# Autodesk Inventor assembly: case
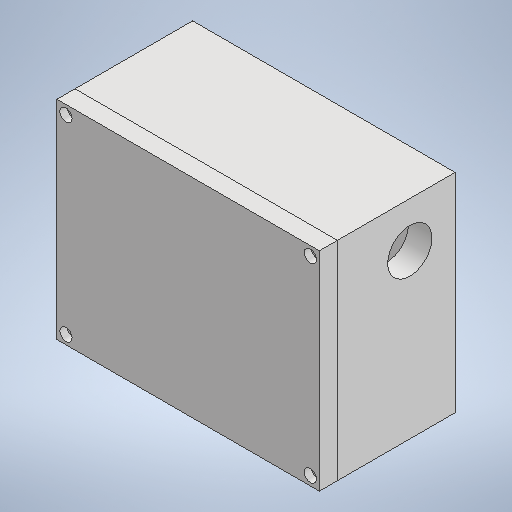
[picture p0: Inventor's stored thumbnail of the model, 512x512]
Saved by Autodesk Inventor 2027 (Build 310192060, 192F)
## iProperties
Created: 2026-06-17
Part Number: case
Document SubType Name: Assembly
Designer: Felix
Author: Felix
## Documents named in this file (3)
- C:\Users\Felix\Dokumente\Git Repos\ACE-II-AdaptiveControl\CAD\case.iam
- C:\Users\Felix\Dokumente\Git Repos\ACE-II-AdaptiveControl\CAD\boden.ipt
- C:\Users\Felix\Dokumente\Git Repos\ACE-II-AdaptiveControl\CAD\schale.ipt
## Components (2 placed, 2 different names)
1. boden:1 — Flush:1, Flush:2, Flush:3, Flush:4
2. schale:1 — Flush:1, Flush:2, Flush:3, Flush:4
## Relationships (4: Flush 4)
- Flush:1: boden:1 ↔ schale:1
- Flush:2: boden:1 ↔ schale:1
- Flush:3: boden:1 ↔ schale:1
- Flush:4: boden:1 ↔ schale:1
